# Autodesk Inventor assembly: assembly
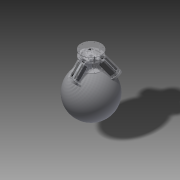
[picture p0: Inventor's stored thumbnail of the model, 180x180]
Saved by Autodesk Inventor 2015 (Build 190159000, 159)
## iProperties
Created: 2015-10-17
Part Number: assembly
Document SubType Name: Assembly
Designer: Brian
Mass: 773.901 g
Surface Area: 3761.23 cm^2
Volume: 5931.58 cm^3
Density: 0.130471 g/cm^3
Author: Brian
## Documents named in this file (14)
- D:\Brian\Dropbox\Brian\Other\balancing things\ballbot\assembly.iam
- D:\Brian\Dropbox\Brian\Other\balancing things\ballbot\motor mount side.ipt
- D:\Brian\Dropbox\Brian\Other\balancing things\ballbot\motor mount.ipt
- D:\Brian\Dropbox\Brian\Other\balancing things\ballbot\B72EB14AA30C\B72EB14AA30C.iam
- D:\Brian\Dropbox\Brian\Other\balancing things\ballbot\motor holder.ipt
- D:\Brian\Dropbox\Brian\Other\balancing things\ballbot\soccer ball.ipt
- D:\Brian\Dropbox\Brian\Other\balancing things\ballbot\wheel.ipt
- D:\Brian\Dropbox\Brian\Other\balancing things\ballbot\motor mount top.ipt
- D:\Brian\Dropbox\Brian\Other\balancing things\ballbot\core2.ipt
- D:\Brian\Dropbox\Brian\Other\balancing things\ballbot\top plate.ipt
- D:\Brian\Dropbox\Brian\Other\balancing things\ballbot\bottom plate.ipt
- D:\Brian\Dropbox\Brian\Other\balancing things\ballbot\18650.ipt
- D:\Brian\Dropbox\Brian\Other\balancing things\ballbot\top top plate.ipt
- D:\Brian\Dropbox\Brian\Other\balancing things\ballbot\spacer.ipt
## Components (33 placed, 13 different names)
1. soccer ball:1 — Tangent:1, Mate:11, Mate:13
2. core2:1 — Mate:10, Mate:11, Flush:5, Mate:14, Mate:15, Mate:16
3. top plate:1 — Mate:14, Mate:15, Angle:1, Mate:18, Flush:7, Flush:8, Mate:27, Mate:28, Mate:29, Mate:30, Mate:31, Mate:32
4. bottom plate:1 — Mate:16, Mate:17, Mate:18
5. 18650:1 — Tangent:2, Flush:6
6. top top plate:1 — Flush:7, Flush:8, Mate:33
7. spacer:1 — Mate:29, Mate:30, Mate:33
8. spacer:3 — Mate:31, Mate:32
9. spacer:4 — Mate:27, Mate:28
10. motor mount top:1 — Mate:7, Mate:8, Mate:9, Angle:1, Mate:19, Mate:20, Mate:21, Tangent:2, Flush:6
11. motor mount side:1 — Mate:1, Flush:2, Flush:3, Mate:5, Mate:7, Mate:10, Flush:5, Mate:17
12. motor mount side:2 — Mate:19, Mate:20, Mate:21, Mate:23
13. motor holder:2 — Mate:22, Mate:23, Mate:24
14. motor holder:1 — Mate:5, Mate:25, Mate:26
15. motor mount:1 — Mate:1, Flush:2, Flush:3, Mate:2, Mate:3, Mate:8, Mate:9, Mate:12, Mate:24, Mate:25
16. wheel:1 — Mate:6, Tangent:1, Mate:12, Mate:13
17. B72EB14AA30C:1 [sub-assembly] — Mate:2, Mate:3, Mate:6, Mate:22, Mate:26
18. motor mount top:2
19. motor mount side:3
20. motor mount side:4
21. motor holder:3
22. motor holder:4
23. motor mount:2
24. wheel:2
25. B72EB14AA30C:2 [sub-assembly]
26. motor mount top:3
27. motor mount side:5
28. motor mount side:6
29. motor holder:5
30. motor holder:6
31. motor mount:3
32. wheel:3
33. B72EB14AA30C:3 [sub-assembly]
## Component patterns: (3 elements, first: motor mount top:1 + motor mount side:1 + motor mount side:2 + motor holder:2 + motor holder:1 + motor mount:1 + wheel:1 + B72EB14AA30C:1)
## Relationships (41: Mate 32, Flush 6, Tangent 2, Angle 1)
- Mate:1: motor mount side:1 ↔ motor mount:1
- Flush:2: motor mount side:1 ↔ motor mount:1
- Flush:3: motor mount side:1 ↔ motor mount:1
- Mate:2: motor mount:1 ↔ B72EB14AA30C:1
- Mate:3: motor mount:1 ↔ B72EB14AA30C:1
- Mate:5: motor mount side:1 ↔ motor holder:1
- Mate:6: wheel:1 ↔ B72EB14AA30C:1
- Tangent:1: soccer ball:1 ↔ wheel:1
- Mate:7: motor mount top:1 ↔ motor mount side:1
- Mate:8: motor mount top:1 ↔ motor mount:1
- Mate:9: motor mount top:1 ↔ motor mount:1
- Mate:10: core2:1 ↔ motor mount side:1
- Mate:11: soccer ball:1 ↔ core2:1
- Mate:12 (4 mm): motor mount:1 ↔ wheel:1
- Flush:5: core2:1 ↔ motor mount side:1
- Mate:13: soccer ball:1 ↔ wheel:1
- Mate:14: core2:1 ↔ top plate:1
- Mate:15: core2:1 ↔ top plate:1
- Angle:1 (180 deg): top plate:1 ↔ motor mount top:1
- Mate:16: core2:1 ↔ bottom plate:1
- Mate:17: bottom plate:1 ↔ motor mount side:1
- Mate:18: top plate:1 ↔ bottom plate:1
- Mate:19: motor mount top:1 ↔ motor mount side:2
- Mate:20: motor mount top:1 ↔ motor mount side:2
- Mate:21: motor mount top:1 ↔ motor mount side:2
- Mate:22: motor holder:2 ↔ B72EB14AA30C:1
- Mate:23: motor mount side:2 ↔ motor holder:2
- Mate:24: motor holder:2 ↔ motor mount:1
- Mate:25: motor holder:1 ↔ motor mount:1
- Mate:26: motor holder:1 ↔ B72EB14AA30C:1
- Tangent:2: 18650:1 ↔ motor mount top:1
- Flush:6 (15 mm): 18650:1 ↔ motor mount top:1
- Flush:7: top plate:1 ↔ top top plate:1
- Flush:8: top plate:1 ↔ top top plate:1
- Mate:27: top plate:1 ↔ spacer:4
- Mate:28: top plate:1 ↔ spacer:4
- Mate:29: top plate:1 ↔ spacer:1
- Mate:30: top plate:1 ↔ spacer:1
- Mate:31: top plate:1 ↔ spacer:3
- Mate:32: top plate:1 ↔ spacer:3
- Mate:33: top top plate:1 ↔ spacer:1
